# Autodesk Inventor assembly: AssemblyNEWarm
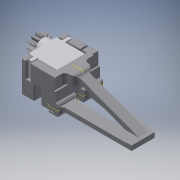
[picture p0: Inventor's stored thumbnail of the model, 180x180]
Saved by Autodesk Inventor 2018 (Build 220112000, 112)
## iProperties
Created: 2017-12-09
Part Number: AssemblyNEWarm
Document SubType Name: Assembly
Designer: kcmat
Author: kcmat
## Documents named in this file (7)
- C:\Users\reide\OneDrive\Documents\Inventor\TSA\2018\Animatronics\Tortoise\arms\AssemblyNEWarm.iam
- C:\Users\reide\OneDrive\Documents\Inventor\TSA\2018\Animatronics\Tortoise\arms\newShoulder.ipt
- C:\Users\reide\OneDrive\Documents\Inventor\TSA\2018\Animatronics\Tortoise\arms\straightBar.ipt
- C:\Users\reide\OneDrive\Documents\Inventor\TSA\2018\Animatronics\Tortoise\arms\AngleArm.ipt
- C:\Users\reide\OneDrive\Documents\Inventor\TSA\2018\Animatronics\Tortoise\arms\bottomARM.ipt
- C:\Users\reide\OneDrive\Documents\Inventor\TSA\2018\Animatronics\Tortoise\Mock Parts\servo (2).ipt
- C:\Users\reide\OneDrive\Documents\Inventor\TSA\2018\Animatronics\Tortoise\Pinion final.ipt
## Components (6 placed, 6 different names)
1. newShoulder:1 — Flush:1, Mate:1, Mate:2, Flush:2, Mate:3, Mate:4, Mate:6, Flush:3, Flush:4, Mate:7, Flush:5
2. straightBar:1 — Flush:2, Mate:3, Mate:4
3. AngleArm:1 — Flush:1, Mate:1, Mate:2
4. bottomARM:1 — Mate:6, Flush:3, Flush:4
5. servo (2):2 — Mate:7, Flush:5, Mate:8, Mate:9
6. Pinion final:1 — Mate:8, Mate:9
## Relationships (13: Mate 8, Flush 5)
- Flush:1: newShoulder:1 ↔ AngleArm:1
- Mate:1: newShoulder:1 ↔ AngleArm:1
- Mate:2: newShoulder:1 ↔ AngleArm:1
- Flush:2: newShoulder:1 ↔ straightBar:1
- Mate:3: newShoulder:1 ↔ straightBar:1
- Mate:4: newShoulder:1 ↔ straightBar:1
- Mate:6: newShoulder:1 ↔ bottomARM:1
- Flush:3: newShoulder:1 ↔ bottomARM:1
- Flush:4: newShoulder:1 ↔ bottomARM:1
- Mate:7: newShoulder:1 ↔ servo (2):2
- Flush:5: newShoulder:1 ↔ servo (2):2
- Mate:8: servo (2):2 ↔ Pinion final:1
- Mate:9: servo (2):2 ↔ Pinion final:1
